# Autodesk Inventor assembly: top
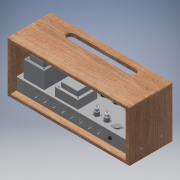
[picture p0: Inventor's stored thumbnail of the model, 180x180]
Saved by Autodesk Inventor 2016 (Build 200138000, 138)
## iProperties
Created: 2015-10-24
Part Number: top
Document SubType Name: Assembly
Designer: jeremyhale
Author: jeremyhale
## Documents named in this file (11)
- \\psf\Home\Documents\Poorhouse\git\p0001\top.iam
- \\psf\Home\Documents\Poorhouse\git\p0001\cabinet.iam
- \\psf\Home\Documents\Poorhouse\git\p0001\chassis.iam
- chassis.iam
- \\psf\Home\Documents\Poorhouse\git\p0001\cabinet-bottom.ipt
- \\psf\Home\Documents\Poorhouse\git\p0001\top\Design Accelerator\Bolted Connection10.iam
- \\psf\Home\Documents\Poorhouse\git\p0001\top\Design Accelerator\Bolted Connection11.iam
- \\psf\Home\Documents\Poorhouse\git\p0001\top\Design Accelerator\Bolted Connection1.iam
- \\psf\Home\Documents\Poorhouse\git\p0001\top\Design Accelerator\Bolted Connection2.iam
- \\psf\Home\Documents\Poorhouse\git\p0001\top\Design Accelerator\Bolted Connection3.iam
- \\psf\Home\Documents\Poorhouse\git\p0001\top\Design Accelerator\Bolted Connection4.iam
## Components (9 placed, 4 different names)
1. cabinet:1 [sub-assembly] — Flush:2, Flush:3, Flush:6, Flush:8, Flush:9, Mate:14, Mate:57, Mate:59
2. chassis:1 [sub-assembly] — Mate:1, Flush:4, Flush:5, Mate:58, Mate:60, Mate:62, Mate:64, Mate:66, Mate:68
3. cabinet-bottom:1 — Mate:1, Flush:4, Flush:5, Flush:6, Flush:8, Flush:9, Mate:14, Mate:61, Mate:63, Mate:65, Mate:67
4. Bolted Connection:5 [sub-assembly] — Mate:57, Mate:58
5. Bolted Connection:6 [sub-assembly] — Mate:59, Mate:60
6. Bolted Connection:7 [sub-assembly] — Mate:61, Mate:62
7. Bolted Connection:8 [sub-assembly] — Mate:63, Mate:64
8. Bolted Connection:9 [sub-assembly] — Mate:65, Mate:66
9. Bolted Connection:10 [sub-assembly] — Mate:67, Mate:68
## Relationships (21: Mate 14, Flush 7)
- Flush:2: cabinet:1
- Flush:3: cabinet:1
- Mate:1: chassis:1 ↔ cabinet-bottom:1
- Flush:4 (-25.4 mm): chassis:1 ↔ cabinet-bottom:1
- Flush:5: chassis:1 ↔ cabinet-bottom:1
- Flush:6: cabinet:1 ↔ cabinet-bottom:1
- Flush:8: cabinet:1 ↔ cabinet-bottom:1
- Flush:9: cabinet:1 ↔ cabinet-bottom:1
- Mate:14: cabinet:1 ↔ cabinet-bottom:1
- Mate:57: cabinet:1 ↔ Bolted Connection:5
- Mate:58: chassis:1 ↔ Bolted Connection:5
- Mate:59: cabinet:1 ↔ Bolted Connection:6
- Mate:60: chassis:1 ↔ Bolted Connection:6
- Mate:61: cabinet-bottom:1 ↔ Bolted Connection:7
- Mate:62: chassis:1 ↔ Bolted Connection:7
- Mate:63: cabinet-bottom:1 ↔ Bolted Connection:8
- Mate:64: chassis:1 ↔ Bolted Connection:8
- Mate:65: cabinet-bottom:1 ↔ Bolted Connection:9
- Mate:66: chassis:1 ↔ Bolted Connection:9
- Mate:67: cabinet-bottom:1 ↔ Bolted Connection:10
- Mate:68: chassis:1 ↔ Bolted Connection:10
